# Autodesk Inventor assembly: FullView
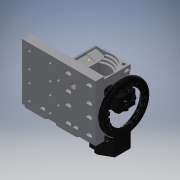
[picture p0: Inventor's stored thumbnail of the model, 180x180]
Saved by Autodesk Inventor 2019 (Build 230136000, 136)
## iProperties
Created: 2018-06-29
Part Number: FullView
Material: Ogólny
Document SubType Name: Assembly
Designer: Kamil
Author: Kamil
## Documents named in this file (7)
- D:\Git\3DPrinting\E3DExtruderHolder\FullView.iam
- D:\Git\3DPrinting\E3DExtruderHolder\ExtruderHolder.ipt
- D:\Git\3DPrinting\E3DExtruderHolder\ExtruderCooler.ipt
- D:\Git\3DPrinting\E3DExtruderHolder\ExtruderClamp.ipt
- D:\Git\3DPrinting\E3DExtruderHolder\FanV2_Shorter.ipt
- D:\Git\3DPrinting\E3DExtruderHolder\BlowerFan.ipt
- D:\Git\3DPrinting\E3DExtruderHolder\E3D_v6_To_Spec.ipt
## Components (6 placed, 6 different names)
1. ExtruderCooler:1
2. ExtruderClamp:1 — Walcowe:1
3. ExtruderHolder:1 — Walcowe:1, Obrotowe:1, Obrotowe:2
4. FanV2_Shorter:1
5. BlowerFan:1 — Obrotowe:1
6. E3D_v6_To_Spec:1 — Obrotowe:2
## Relationships (3: RevoluteJoint 2, CylindricalJoint 1)
- Walcowe:1 [CylindricalJoint]: ExtruderClamp:1 ↔ ExtruderHolder:1
- Obrotowe:1 [RevoluteJoint] (-3 mm): ExtruderHolder:1 ↔ BlowerFan:1
- Obrotowe:2 [RevoluteJoint]: ExtruderHolder:1 ↔ E3D_v6_To_Spec:1
